# Autodesk Inventor assembly: nano cam assy
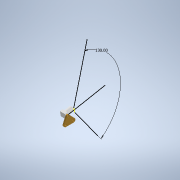
[picture p0: Inventor's stored thumbnail of the model, 180x180]
Saved by Autodesk Inventor 2020 (Build 240168000, 168)
## iProperties
Created: 2022-05-06
Part Number: nano cam assy
Document SubType Name: Assembly
Designer: Steven
Author: Steven
## Documents named in this file (3)
- Y:\FPV drone stuff\0 Street League\Frames\PB-Kauri-X\3D prints\35 mm canopy\work in progress prints\nano cam assy.iam
- Y:\FPV drone stuff\0 Street League\Frames\PB-Kauri-X\3D prints\35 mm canopy\work in progress prints\Kauri modular camera mount nano cam.ipt
- Y:\FPV drone stuff\0 Street League\Frames\PB-Kauri-X\3D prints\35 mm canopy\work in progress prints\HDzero runcam nano spacer.ipt
## Components (2 placed, 2 different names)
1. Kauri modular camera mount nano cam:1 — Mate:1, Mate:2, Tangent:1, Insert:1
2. HDzero runcam nano spacer:1 — Insert:1
## Relationships (4: Mate 2, Tangent 1, Insert 1)
- Mate:1: Kauri modular camera mount nano cam:1
- Mate:2: Kauri modular camera mount nano cam:1
- Tangent:1: Kauri modular camera mount nano cam:1
- Insert:1: Kauri modular camera mount nano cam:1 ↔ HDzero runcam nano spacer:1
